# Autodesk Inventor assembly: main_flap
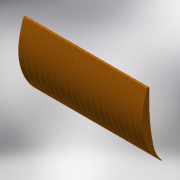
[picture p0: Inventor's stored thumbnail of the model, 180x180]
Saved by Autodesk Inventor 2018.2 (Build 222227000, 227)
## iProperties
Created: 2017-12-11
Part Number: main_flap
Material: 一般
Document SubType Name: Assembly
Designer: kuwano
Mass: 28711.4 g
Surface Area: 25647 cm^2
Volume: 23370.8 cm^3
Density: 1.22852 g/cm^3
Author: kuwano
## Documents named in this file (5)
- D:\kuwano\Documents\Inventor\KITformula\AeroCAD2018\CAD\Inventor\製作用CAD\R-wing\parts\main_flap\main_flap.iam
- D:\kuwano\Documents\Inventor\KITformula\AeroCAD2018\CAD\Inventor\製作用CAD\R-wing\parts\main_flap\parts\styro_50_main.ipt
- D:\kuwano\Documents\Inventor\KITformula\AeroCAD2018\CAD\Inventor\製作用CAD\R-wing\parts\main_flap\parts\pipe.ipt
- D:\kuwano\Documents\Inventor\KITformula\AeroCAD2018\CAD\Inventor\製作用CAD\R-wing\parts\main_flap\parts\pipe_square.ipt
- D:\kuwano\Documents\Inventor\KITformula\AeroCAD2018\CAD\Inventor\製作用CAD\R-wing\parts\main_flap\parts\pipe_square_back.ipt
## Components (25 placed, 4 different names)
1. styro_50_main:1 — メイト:1, メイト:2, メイト:29, フラッシュ:1, フラッシュ:2
2. styro_50_main:2 — メイト:1, メイト:2, メイト:3, メイト:4, メイト:29, メイト:30
3. styro_50_main:3 — メイト:3, メイト:4, メイト:5, メイト:6, メイト:30, メイト:31
4. styro_50_main:4 — メイト:5, メイト:6, メイト:31, メイト:43, メイト:44, メイト:50, メイト:67
5. styro_50_main:5 — メイト:43, メイト:44, メイト:49, メイト:62, メイト:67
6. styro_50_main:6 — メイト:7, メイト:8, メイト:32, メイト:62
7. styro_50_main:7 — メイト:7, メイト:8, メイト:9, メイト:10, メイト:32, メイト:33
8. styro_50_main:8 — メイト:9, メイト:10, メイト:11, メイト:12, メイト:33, メイト:34
9. styro_50_main:9 — メイト:11, メイト:12, メイト:13, メイト:34, メイト:35, メイト:65, メイト:71
10. styro_50_main:10 — メイト:13, メイト:16, メイト:35, メイト:36, メイト:65, メイト:66
11. styro_50_main:11 — メイト:16, メイト:17, メイト:18, メイト:36, メイト:37, メイト:66, メイト:72
12. styro_50_main:12 — メイト:17, メイト:18, メイト:19, メイト:20, メイト:37, メイト:38
13. styro_50_main:13 — メイト:19, メイト:20, メイト:21, メイト:22, メイト:38, メイト:39
14. styro_50_main:14 — メイト:21, メイト:22, メイト:39, メイト:45, メイト:46, メイト:49, メイト:52, メイト:61
15. styro_50_main:15 — メイト:45, メイト:46, メイト:47, メイト:48, メイト:61, メイト:68
16. styro_50_main:16 — メイト:23, メイト:24, メイト:40, メイト:68
17. styro_50_main:17 — メイト:23, メイト:24, メイト:25, メイト:26, メイト:40, メイト:41
18. styro_50_main:18 — メイト:25, メイト:26, メイト:27, メイト:28, メイト:41, メイト:42
19. styro_50_main:19 — メイト:27, メイト:28, メイト:42, メイト:47, メイト:48, フラッシュ:3, フラッシュ:4, メイト:54
20. pipe:1 — フラッシュ:2, フラッシュ:4, メイト:54, メイト:73, メイト:74
21. pipe:2 — メイト:50, フラッシュ:1, メイト:52, メイト:53, フラッシュ:3, フラッシュ:8, メイト:69, メイト:70
22. pipe_square:1 — メイト:70, フラッシュ:9, 角度:1, メイト:71, フラッシュ:10
23. pipe_square:2 — メイト:69, フラッシュ:9, メイト:72, フラッシュ:11
24. pipe_square_back:1 — メイト:73, フラッシュ:10, フラッシュ:12
25. pipe_square_back:2 — メイト:74, フラッシュ:11, フラッシュ:12
## Relationships (73: Mate 63, Flush 9, Angle 1)
- メイト:1 [Mate]: styro_50_main:1 ↔ styro_50_main:2
- メイト:2 [Mate]: styro_50_main:1 ↔ styro_50_main:2
- メイト:3 [Mate]: styro_50_main:2 ↔ styro_50_main:3
- メイト:4 [Mate]: styro_50_main:2 ↔ styro_50_main:3
- メイト:5 [Mate]: styro_50_main:3 ↔ styro_50_main:4
- メイト:6 [Mate]: styro_50_main:3 ↔ styro_50_main:4
- メイト:7 [Mate]: styro_50_main:6 ↔ styro_50_main:7
- メイト:8 [Mate]: styro_50_main:6 ↔ styro_50_main:7
- メイト:9 [Mate]: styro_50_main:7 ↔ styro_50_main:8
- メイト:10 [Mate]: styro_50_main:7 ↔ styro_50_main:8
- メイト:11 [Mate]: styro_50_main:8 ↔ styro_50_main:9
- メイト:12 [Mate]: styro_50_main:8 ↔ styro_50_main:9
- メイト:13 [Mate]: styro_50_main:9 ↔ styro_50_main:10
- メイト:16 [Mate]: styro_50_main:10 ↔ styro_50_main:11
- メイト:17 [Mate]: styro_50_main:11 ↔ styro_50_main:12
- メイト:18 [Mate]: styro_50_main:11 ↔ styro_50_main:12
- メイト:19 [Mate]: styro_50_main:12 ↔ styro_50_main:13
- メイト:20 [Mate]: styro_50_main:12 ↔ styro_50_main:13
- メイト:21 [Mate]: styro_50_main:13 ↔ styro_50_main:14
- メイト:22 [Mate]: styro_50_main:13 ↔ styro_50_main:14
- メイト:23 [Mate]: styro_50_main:16 ↔ styro_50_main:17
- メイト:24 [Mate]: styro_50_main:16 ↔ styro_50_main:17
- メイト:25 [Mate]: styro_50_main:17 ↔ styro_50_main:18
- メイト:26 [Mate]: styro_50_main:17 ↔ styro_50_main:18
- メイト:27 [Mate]: styro_50_main:18 ↔ styro_50_main:19
- メイト:28 [Mate]: styro_50_main:18 ↔ styro_50_main:19
- メイト:29 [Mate]: styro_50_main:1 ↔ styro_50_main:2
- メイト:30 [Mate]: styro_50_main:2 ↔ styro_50_main:3
- メイト:31 [Mate]: styro_50_main:3 ↔ styro_50_main:4
- メイト:32 [Mate]: styro_50_main:6 ↔ styro_50_main:7
- メイト:33 [Mate]: styro_50_main:7 ↔ styro_50_main:8
- メイト:34 [Mate]: styro_50_main:8 ↔ styro_50_main:9
- メイト:35 [Mate]: styro_50_main:9 ↔ styro_50_main:10
- メイト:36 [Mate]: styro_50_main:10 ↔ styro_50_main:11
- メイト:37 [Mate]: styro_50_main:11 ↔ styro_50_main:12
- メイト:38 [Mate]: styro_50_main:12 ↔ styro_50_main:13
- メイト:39 [Mate]: styro_50_main:13 ↔ styro_50_main:14
- メイト:40 [Mate]: styro_50_main:16 ↔ styro_50_main:17
- メイト:41 [Mate]: styro_50_main:17 ↔ styro_50_main:18
- メイト:42 [Mate]: styro_50_main:18 ↔ styro_50_main:19
- メイト:43 [Mate]: styro_50_main:4 ↔ styro_50_main:5
- メイト:44 [Mate]: styro_50_main:4 ↔ styro_50_main:5
- メイト:45 [Mate]: styro_50_main:14 ↔ styro_50_main:15
- メイト:46 [Mate]: styro_50_main:14 ↔ styro_50_main:15
- メイト:47 [Mate]: styro_50_main:15 ↔ styro_50_main:19
- メイト:48 [Mate]: styro_50_main:15 ↔ styro_50_main:19
- メイト:49 [Mate]: styro_50_main:5 ↔ styro_50_main:14
- メイト:50 [Mate]: styro_50_main:4 ↔ pipe:2
- フラッシュ:1 [Flush]: styro_50_main:1 ↔ pipe:2
- フラッシュ:2 [Flush]: styro_50_main:1 ↔ pipe:1
- メイト:52 [Mate]: styro_50_main:14 ↔ pipe:2
- メイト:53 [Mate]: pipe:2
- フラッシュ:3 [Flush]: styro_50_main:19 ↔ pipe:2
- フラッシュ:4 [Flush]: styro_50_main:19 ↔ pipe:1
- メイト:54 [Mate]: styro_50_main:19 ↔ pipe:1
- メイト:61 [Mate]: styro_50_main:14 ↔ styro_50_main:15
- メイト:62 [Mate]: styro_50_main:5 ↔ styro_50_main:6
- メイト:65 [Mate]: styro_50_main:9 ↔ styro_50_main:10
- メイト:66 [Mate]: styro_50_main:10 ↔ styro_50_main:11
- メイト:67 [Mate]: styro_50_main:4 ↔ styro_50_main:5
- メイト:68 [Mate]: styro_50_main:15 ↔ styro_50_main:16
- フラッシュ:8 [Flush]: pipe:2
- メイト:69 [Mate]: pipe:2 ↔ pipe_square:2
- メイト:70 [Mate]: pipe:2 ↔ pipe_square:1
- フラッシュ:9 [Flush]: pipe_square:1 ↔ pipe_square:2
- 角度:1 [Angle] (0 deg): pipe_square:1
- メイト:71 [Mate] (20 mm): styro_50_main:9 ↔ pipe_square:1
- メイト:72 [Mate] (-20 mm): styro_50_main:11 ↔ pipe_square:2
- メイト:73 [Mate]: pipe:1 ↔ pipe_square_back:1
- メイト:74 [Mate]: pipe:1 ↔ pipe_square_back:2
- フラッシュ:10 [Flush]: pipe_square:1 ↔ pipe_square_back:1
- フラッシュ:11 [Flush]: pipe_square:2 ↔ pipe_square_back:2
- フラッシュ:12 [Flush]: pipe_square_back:1 ↔ pipe_square_back:2
